# Autodesk Inventor assembly: Infill3DExtruder
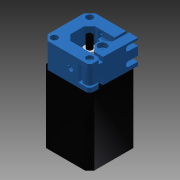
[picture p0: Inventor's stored thumbnail of the model, 180x180]
Saved by Autodesk Inventor 2015 SP1 (Build 190203100, 203)
## iProperties
Created: 2015-04-27
Part Number: Infill3DExtruder
Document SubType Name: Assembly
Designer: Jack
Author: Jack
## Documents named in this file (6)
- C:\Users\Jack\ownCloud\Projects\CrossBot\InventorModel\Extruder\Infill3DExtruder\Infill3DExtruder.iam
- C:\Users\Jack\ownCloud\Projects\CrossBot\InventorModel\Extruder\Infill3DExtruder\Infill3DBody.ipt
- C:\Users\Jack\ownCloud\Projects\CrossBot\InventorModel\Electronics\Motors\StepperMotorNema17x60mm.ipt
- C:\Users\Jack\ownCloud\Projects\CrossBot\InventorModel\Hardware\Extruder\DriveGearMK8.ipt
- C:\Users\Jack\ownCloud\Projects\CrossBot\InventorModel\Extruder\Infill3DExtruder\Infill3DIdler.ipt
- C:\Users\Jack\ownCloud\Projects\CrossBot\InventorModel\Hardware\Bearing\BearingRadialBall\BearingRadialBall624zz.ipt
## Components (5 placed, 5 different names)
1. Infill3DBody:1 — Mate:1, Mate:2, Mate:6, Mate:7, Mate:8
2. StepperMotorNema17x60mm:1 — Mate:1, Mate:2, Mate:4, Mate:5, Mate:6
3. DriveGearMK8:1 — Mate:4, Mate:5
4. Infill3DIdler:1 — Mate:7, Mate:8, Mate:9, Mate:10
5. BearingRadialBall624zz:1 — Mate:9, Mate:10
## Relationships (9: Mate 9)
- Mate:1: Infill3DBody:1 ↔ StepperMotorNema17x60mm:1
- Mate:2: Infill3DBody:1 ↔ StepperMotorNema17x60mm:1
- Mate:4: StepperMotorNema17x60mm:1 ↔ DriveGearMK8:1
- Mate:5 (1 mm): StepperMotorNema17x60mm:1 ↔ DriveGearMK8:1
- Mate:6: Infill3DBody:1 ↔ StepperMotorNema17x60mm:1
- Mate:7: Infill3DBody:1 ↔ Infill3DIdler:1
- Mate:8 (0.2 mm): Infill3DBody:1 ↔ Infill3DIdler:1
- Mate:9: Infill3DIdler:1 ↔ BearingRadialBall624zz:1
- Mate:10: Infill3DIdler:1 ↔ BearingRadialBall624zz:1
